# Autodesk Inventor assembly: Gearbox_Rev_1.0
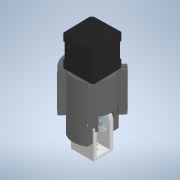
[picture p0: Inventor's stored thumbnail of the model, 180x180]
Saved by Autodesk Inventor 2022 (Build 260153000, 153)
## iProperties
Created: 2022-04-03
Part Number: Gearbox_Rev_1.0
Document SubType Name: Assembly
Designer: Mlees
Author: Mlees
## Documents named in this file (14)
- C:\Users\Mlees\Desktop\504Engineering\Project_0000\Designs\Design_1\Gearbox_Rev_1.0.iam
- C:\Users\Mlees\Desktop\504Engineering\Project_0000\Designs\Design_1\Downloaded_Parts\Nema 17.ipt
- C:\Users\Mlees\Desktop\504Engineering\Project_0000\Designs\Design_1\Created_Parts\96_Teeth_Gear.ipt
- C:\Users\Mlees\Desktop\504Engineering\Project_0000\Designs\Design_1\Created_Parts\96_Teeth_Gear_No_Motor_Mount_2.ipt
- C:\Users\Mlees\Desktop\504Engineering\Project_0000\Designs\Design_1\Downloaded_Parts\Stainless Steel Pan Head Phillips Screws_m2.5x8mm.ipt
- C:\Users\Mlees\Desktop\504Engineering\Project_0000\Designs\Design_1\Created_Parts\24_Teeth_Sun_Gear.ipt
- C:\Users\Mlees\Desktop\504Engineering\Project_0000\Designs\Design_1\Created_Parts\36_Teeth_Planet_Gear.ipt
- C:\Users\Mlees\Desktop\504Engineering\Project_0000\Designs\Design_1\Created_Parts\Planet_Carrier_Mod_1.ipt
- C:\Users\Mlees\Desktop\504Engineering\Project_0000\Designs\Design_1\Created_Parts\Spiral Bevel gear Z2.ipt
- C:\Users\Mlees\Desktop\504Engineering\Project_0000\Designs\Design_1\Created_Parts\Base_Mount.ipt
- C:\Users\Mlees\Desktop\504Engineering\Project_0000\Designs\Design_1\Created_Parts\Lid_Tilt_1.ipt
- C:\Users\Mlees\Desktop\504Engineering\Project_0000\Designs\Design_1\Created_Parts\Lid_Tilt_2.ipt
- C:\Users\Mlees\Desktop\504Engineering\Project_0000\Designs\Design_1\Downloaded_Parts\5972K222_Ball Bearing.ipt
- C:\Users\Mlees\Desktop\504Engineering\Project_0000\Designs\Design_1\Created_Parts\Gearbox_Output.ipt
## Components (28 placed, 13 different names)
1. Nema 17:1 — Rigid:1, Rotational:5
2. 96_Teeth_Gear:1 — Mate:11, Mate:12, Mate:13, Mate:14, Mate:15, Mate:16, Mate:17, Mate:18, Rigid:1, Rigid:2
3. 96_Teeth_Gear_No_Motor_Mount_2:1 — Rigid:2, Rigid:3
4. 96_Teeth_Gear_No_Motor_Mount_2:2 — Rigid:3, Mate:22, Mate:23, Mate:24, Rotational:22, Rotational:23
5. Stainless Steel Pan Head Phillips Screws_m2.5x8mm:1 — Mate:13, Mate:17
6. Stainless Steel Pan Head Phillips Screws_m2.5x8mm:2 — Mate:14, Mate:16
7. Stainless Steel Pan Head Phillips Screws_m2.5x8mm:3 — Mate:12, Mate:18
8. Stainless Steel Pan Head Phillips Screws_m2.5x8mm:4 — Mate:11, Mate:15
9. 24_Teeth_Sun_Gear:1 — Rotational:5, Rotational:9
10. 36_Teeth_Planet_Gear:1 — Rotational:10
11. 36_Teeth_Planet_Gear:2 — Rotational:12
12. 36_Teeth_Planet_Gear:3 — Rotational:11
13. Planet_Carrier_Mod_1:1 — Rotational:9, Rotational:10, Rotational:11, Rotational:12, Rotational:13
14. 36_Teeth_Planet_Gear:4 — Rotational:14
15. 36_Teeth_Planet_Gear:5 — Rotational:15
16. 36_Teeth_Planet_Gear:6 — Rotational:16
17. Planet_Carrier_Mod_1:2 — Rotational:13, Rotational:14, Rotational:15, Rotational:16, Rotational:24
18. 36_Teeth_Planet_Gear:7
19. 36_Teeth_Planet_Gear:8
20. 36_Teeth_Planet_Gear:9
21. Spiral Bevel gear Z2:1 — Mate:19, Mate:20, Mate:21
22. Base_Mount:1 — Mate:19, Mate:20, Mate:21, Mate:32, Mate:33
23. Lid_Tilt_1:1 — Mate:22, Mate:23, Mate:24, Mate:28, Mate:29
24. Lid_Tilt_2:1 — Rotational:22, Rotational:23, Mate:30, Mate:31
25. 5972K222_Ball Bearing:1 — Mate:28, Mate:29
26. 5972K222_Ball Bearing:2 — Mate:30, Mate:31
27. Spiral Bevel gear Z2:2 — Mate:32, Mate:33
28. Gearbox_Output:1 — Rotational:24
## Relationships (35: Mate 20, RevoluteJoint 12, WeldJoint 3)
- Mate:11: 96_Teeth_Gear:1 ↔ Stainless Steel Pan Head Phillips Screws_m2.5x8mm:4
- Mate:12: 96_Teeth_Gear:1 ↔ Stainless Steel Pan Head Phillips Screws_m2.5x8mm:3
- Mate:13: 96_Teeth_Gear:1 ↔ Stainless Steel Pan Head Phillips Screws_m2.5x8mm:1
- Mate:14: 96_Teeth_Gear:1 ↔ Stainless Steel Pan Head Phillips Screws_m2.5x8mm:2
- Mate:15: 96_Teeth_Gear:1 ↔ Stainless Steel Pan Head Phillips Screws_m2.5x8mm:4
- Mate:16: 96_Teeth_Gear:1 ↔ Stainless Steel Pan Head Phillips Screws_m2.5x8mm:2
- Mate:17: 96_Teeth_Gear:1 ↔ Stainless Steel Pan Head Phillips Screws_m2.5x8mm:1
- Mate:18: 96_Teeth_Gear:1 ↔ Stainless Steel Pan Head Phillips Screws_m2.5x8mm:3
- Rigid:1 [WeldJoint]: Nema 17:1 ↔ 96_Teeth_Gear:1
- Rigid:2 [WeldJoint]: 96_Teeth_Gear:1 ↔ 96_Teeth_Gear_No_Motor_Mount_2:1
- Rigid:3 [WeldJoint]: 96_Teeth_Gear_No_Motor_Mount_2:1 ↔ 96_Teeth_Gear_No_Motor_Mount_2:2
- Rotational:5 [RevoluteJoint]: Nema 17:1 ↔ 24_Teeth_Sun_Gear:1
- Rotational:9 [RevoluteJoint] (3 mm): 24_Teeth_Sun_Gear:1 ↔ Planet_Carrier_Mod_1:1
- Rotational:10 [RevoluteJoint]: 36_Teeth_Planet_Gear:1 ↔ Planet_Carrier_Mod_1:1
- Rotational:11 [RevoluteJoint]: 36_Teeth_Planet_Gear:3 ↔ Planet_Carrier_Mod_1:1
- Rotational:12 [RevoluteJoint]: 36_Teeth_Planet_Gear:2 ↔ Planet_Carrier_Mod_1:1
- Rotational:13 [RevoluteJoint] (2.5 mm): Planet_Carrier_Mod_1:1 ↔ Planet_Carrier_Mod_1:2
- Rotational:14 [RevoluteJoint]: 36_Teeth_Planet_Gear:4 ↔ Planet_Carrier_Mod_1:2
- Rotational:15 [RevoluteJoint]: 36_Teeth_Planet_Gear:5 ↔ Planet_Carrier_Mod_1:2
- Rotational:16 [RevoluteJoint]: 36_Teeth_Planet_Gear:6 ↔ Planet_Carrier_Mod_1:2
- Mate:19: Spiral Bevel gear Z2:1 ↔ Base_Mount:1
- Mate:20: Spiral Bevel gear Z2:1 ↔ Base_Mount:1
- Mate:21: Spiral Bevel gear Z2:1 ↔ Base_Mount:1
- Mate:22: 96_Teeth_Gear_No_Motor_Mount_2:2 ↔ Lid_Tilt_1:1
- Mate:23: 96_Teeth_Gear_No_Motor_Mount_2:2 ↔ Lid_Tilt_1:1
- Mate:24: 96_Teeth_Gear_No_Motor_Mount_2:2 ↔ Lid_Tilt_1:1
- Rotational:22 [RevoluteJoint]: 96_Teeth_Gear_No_Motor_Mount_2:2 ↔ Lid_Tilt_2:1
- Rotational:23 [RevoluteJoint]: 96_Teeth_Gear_No_Motor_Mount_2:2 ↔ Lid_Tilt_2:1
- Mate:28: Lid_Tilt_1:1 ↔ 5972K222_Ball Bearing:1
- Mate:29: Lid_Tilt_1:1 ↔ 5972K222_Ball Bearing:1
- Mate:30: Lid_Tilt_2:1 ↔ 5972K222_Ball Bearing:2
- Mate:31: Lid_Tilt_2:1 ↔ 5972K222_Ball Bearing:2
- Mate:32: Base_Mount:1 ↔ Spiral Bevel gear Z2:2
- Mate:33: Base_Mount:1 ↔ Spiral Bevel gear Z2:2
- Rotational:24 [RevoluteJoint] (2 mm): Planet_Carrier_Mod_1:2 ↔ Gearbox_Output:1
